# Autodesk Inventor assembly: manipulator
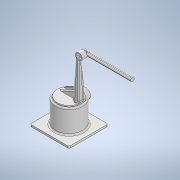
[picture p0: Inventor's stored thumbnail of the model, 180x180]
Saved by Autodesk Inventor 2022.2 (Build 262287010, 287A)
## iProperties
Created: 2022-04-10
Part Number: manipulator
Document SubType Name: Assembly
Designer: stasi
Author: stasi
## Documents named in this file (5)
- D:\stuff\P G\sem6\KPMiR\proj\kpmir\INVENTOR\manipulator.iam
- D:\stuff\P G\sem6\KPMiR\proj\kpmir\INVENTOR\C0.ipt
- D:\stuff\P G\sem6\KPMiR\proj\kpmir\INVENTOR\C1.ipt
- D:\stuff\P G\sem6\KPMiR\proj\kpmir\INVENTOR\C2.ipt
- D:\stuff\P G\sem6\KPMiR\proj\kpmir\INVENTOR\C3.ipt
## Components (4 placed, 4 different names)
1. C0:1 — Flush:1, Flush:3
2. C1:1 — Flush:1, Flush:3, Flush:4, Flush:5
3. C2:1 — Flush:4, Flush:5, Flush:6, Flush:8
4. C3:1 — Flush:6, Flush:8
## Relationships (6: Flush 6)
- Flush:1: C0:1 ↔ C1:1
- Flush:3: C0:1 ↔ C1:1
- Flush:4: C1:1 ↔ C2:1
- Flush:5: C1:1 ↔ C2:1
- Flush:6: C2:1 ↔ C3:1
- Flush:8: C2:1 ↔ C3:1
